# Autodesk Inventor assembly: FIXT1-002_CAM1
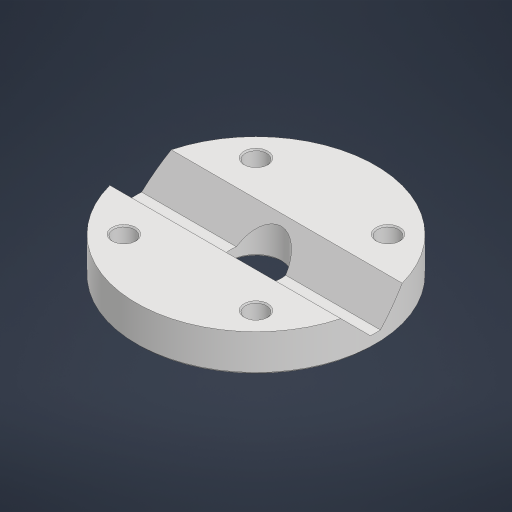
[picture p0: Inventor's stored thumbnail of the model, 512x512]
Saved by Autodesk Inventor 2024.3 (Build 283343000, 343)
## iProperties
Created: 2024-09-25
Part Number: FIXT1-002_CAM1
Document SubType Name: Assembly
Designer: fablabadmin
Author: fablabadmin
## Documents named in this file (8)
- C:\Users\fablabadmin\Documents\_Benjamin_S\_3dCAD\HHVerkstad\Hammer1\_FIXT\_FIXT1-002_CAM1\FIXT1-002_CAM1.iam
- C:\Users\fablabadmin\Documents\_Benjamin_S\_3dCAD\_Config\KemmlerVise\OP1-KemmlerVise.iam
- C:\Users\fablabadmin\Documents\_Benjamin_S\_3dCAD\_Config\KemmlerVise\OP2-KemmlerVise.iam
- C:\Users\fablabadmin\Documents\_Benjamin_S\_3dCAD\HHVerkstad\Hammer1\_FIXT\HM1_FIXT1-002.ipt
- C:\Users\fablabadmin\Documents\_Benjamin_S\_3dCAD\HHVerkstad\Hammer1\_FIXT\_FIXT1-001_CAM1\JawDualSided-Aluminum 6061.ipt
- C:\Users\fablabadmin\Documents\_Benjamin_S\_3dCAD\HHVerkstad\Hammer1\_FIXT\_FIXT1-001_CAM1\JawDualSided-Aluminum 6061MIR.ipt
- C:\Users\fablabadmin\Documents\_Benjamin_S\_3dCAD\HHVerkstad\Hammer1\_FIXT\_FIXT1-002_CAM1\RoundStock.ipt
- C:\Users\fablabadmin\Documents\_Benjamin_S\_3dCAD\_Config\_CAM_SIM\FixtureParts\parallels3mm.xlsx
## Components (8 placed, 6 different names)
1. HM1_FIXT1-002:1 — Mate:8, Tangent:5, Tangent:6, Tangent:7, Tangent:8, Mate:9, Flush:5, Mate:11
2. RoundStock:1 — Mate:9, Flush:5, Mate:10, Tangent:9, Tangent:10, Tangent:11, Tangent:12, Angle:3
3. OP1-KemmlerVise:1 [sub-assembly] — Mate:1, Mate:2, Flush:1, Mate:3, Angle:1
4. JawDualSided-Aluminum 6061:1 — Mate:1, Flush:1, Flush:2, Mate:3, Mate:10, Tangent:9, Tangent:10
5. JawDualSided-Aluminum 6061MIR:1 — Mate:2, Flush:2, Tangent:11, Tangent:12
6. OP2-KemmlerVise:1 [sub-assembly] — Mate:5, Mate:6, Flush:3, Mate:7, Angle:2, Mate:12
7. JawDualSided-Aluminum 6061:2 — Mate:5, Flush:3, Flush:4, Mate:7, Mate:8, Tangent:5, Tangent:6
8. JawDualSided-Aluminum 6061MIR:2 — Mate:6, Flush:4, Tangent:7, Tangent:8
## Relationships (28: Mate 12, Tangent 8, Flush 5, Angle 3)
- Mate:1: OP1-KemmlerVise:1 ↔ JawDualSided-Aluminum 6061:1
- Mate:2: OP1-KemmlerVise:1 ↔ JawDualSided-Aluminum 6061MIR:1
- Flush:1: OP1-KemmlerVise:1 ↔ JawDualSided-Aluminum 6061:1
- Flush:2: JawDualSided-Aluminum 6061:1 ↔ JawDualSided-Aluminum 6061MIR:1
- Mate:3: OP1-KemmlerVise:1 ↔ JawDualSided-Aluminum 6061:1
- Mate:5: OP2-KemmlerVise:1 ↔ JawDualSided-Aluminum 6061:2
- Mate:6: OP2-KemmlerVise:1 ↔ JawDualSided-Aluminum 6061MIR:2
- Flush:3: OP2-KemmlerVise:1 ↔ JawDualSided-Aluminum 6061:2
- Flush:4: JawDualSided-Aluminum 6061:2 ↔ JawDualSided-Aluminum 6061MIR:2
- Mate:7: OP2-KemmlerVise:1 ↔ JawDualSided-Aluminum 6061:2
- Mate:8: HM1_FIXT1-002:1 ↔ JawDualSided-Aluminum 6061:2
- Tangent:5: HM1_FIXT1-002:1 ↔ JawDualSided-Aluminum 6061:2
- Tangent:6: HM1_FIXT1-002:1 ↔ JawDualSided-Aluminum 6061:2
- Tangent:7: HM1_FIXT1-002:1 ↔ JawDualSided-Aluminum 6061MIR:2
- Tangent:8: HM1_FIXT1-002:1 ↔ JawDualSided-Aluminum 6061MIR:2
- Angle:1 (0 deg): OP1-KemmlerVise:1
- Angle:2 (0 deg): OP2-KemmlerVise:1
- Mate:9: HM1_FIXT1-002:1 ↔ RoundStock:1
- Flush:5 (-4 mm): HM1_FIXT1-002:1 ↔ RoundStock:1
- Mate:10: RoundStock:1 ↔ JawDualSided-Aluminum 6061:1
- Tangent:9: RoundStock:1 ↔ JawDualSided-Aluminum 6061:1
- Tangent:10: RoundStock:1 ↔ JawDualSided-Aluminum 6061:1
- Tangent:11: RoundStock:1 ↔ JawDualSided-Aluminum 6061MIR:1
- Tangent:12: RoundStock:1 ↔ JawDualSided-Aluminum 6061MIR:1
- Angle:3 (0 deg): RoundStock:1
- Mate:11: HM1_FIXT1-002:1
- Mate:12: OP2-KemmlerVise:1
- Mate:13
## Named parameters: PRL13 = 13 mm, PRL16 = 16 mm, PRL19 = 19 mm, PRL22 = 22 mm, PRL28 = 28 mm, PRL31 = 31 mm, PRL35 = 35 mm, PRL38 = 38 mm, PRL41 = 41 mm
